# Autodesk Inventor assembly: pcb_assembly
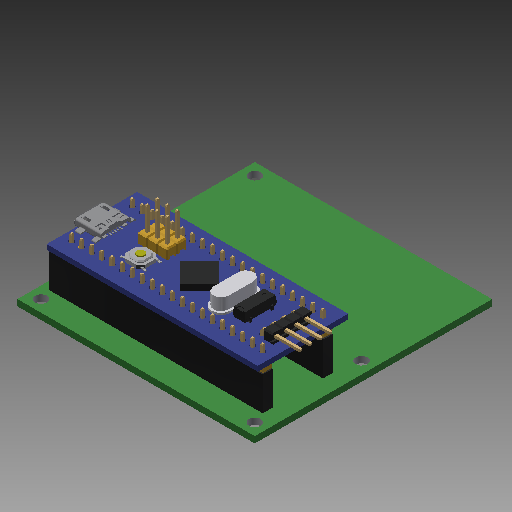
[picture p0: Inventor's stored thumbnail of the model, 512x512]
Saved by Autodesk Inventor 2018 (Build 220112000, 112)
## iProperties
Created: 2018-12-04
Part Number: pcb_assembly
Document SubType Name: Assembly
Designer: jaspe
Author: jaspe
## Documents named in this file (4)
- C:\Users\jaspe\bitbots_hardware\wolfgang\assembly\legs\foot\pcb_assembly.iam
- C:\Users\jaspe\bitbots_hardware\wolfgang\assembly\legs\foot\bluepill\STM32F103C8T6_Blue_Pill v6.iam
- C:\Users\jaspe\bitbots_hardware\wolfgang\assembly\legs\foot\forcefoot_pcb.ipt
- C:\Users\jaspe\bitbots_hardware\wolfgang\assembly\legs\foot\socket_pcb.ipt
## Components (4 placed, 3 different names)
1. STM32F103C8T6_Blue_Pill v6:1 [sub-assembly] — Flush:4, Flush:5, Mate:2, Mate:3, Flush:6
2. forcefoot_pcb:1 — Flush:1, Flush:2, Flush:3, Mate:1
3. socket_pcb:1 — Flush:2, Mate:3, Flush:6
4. socket_pcb:2 — Flush:1, Flush:3, Mate:1, Flush:4, Flush:5, Mate:2
## Relationships (9: Flush 6, Mate 3)
- Flush:1 (4 mm): forcefoot_pcb:1 ↔ socket_pcb:2
- Flush:2 (4 mm): forcefoot_pcb:1 ↔ socket_pcb:1
- Flush:3 (6 mm): forcefoot_pcb:1 ↔ socket_pcb:2
- Mate:1: forcefoot_pcb:1 ↔ socket_pcb:2
- Flush:4: STM32F103C8T6_Blue_Pill v6:1 ↔ socket_pcb:2
- Flush:5: STM32F103C8T6_Blue_Pill v6:1 ↔ socket_pcb:2
- Mate:2: STM32F103C8T6_Blue_Pill v6:1 ↔ socket_pcb:2
- Mate:3: STM32F103C8T6_Blue_Pill v6:1 ↔ socket_pcb:1
- Flush:6: STM32F103C8T6_Blue_Pill v6:1 ↔ socket_pcb:1
